# Autodesk Inventor assembly: AGf
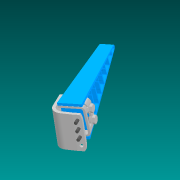
[picture p0: Inventor's stored thumbnail of the model, 180x180]
Saved by Autodesk Inventor 2020.3 (Build 243373000, 373)
## iProperties
Created: 2020-05-25
Part Number: AGf
Document SubType Name: Assembly
Designer: Svend
Author: Svend
## Documents named in this file (4)
- C:\Users\Svend\OneDrive\Documents\GitHub\BeerMinder\3D-model\gripper\AGf.iam
- C:\Users\Svend\OneDrive\Documents\GitHub\BeerMinder\3D-model\servo\AIS2020\3899099 DHAS-MA-B6-80.iam
- C:\Users\Svend\OneDrive\Documents\GitHub\BeerMinder\3D-model\servo\AIS2020\4463570 DHAS-ME-H9-80.iam
- C:\Users\Svend\OneDrive\Documents\GitHub\BeerMinder\3D-model\servo\3998964 DHAS-GF-80-U-BU.ipt
## Components (3 placed, 3 different names)
1. 3899099 DHAS-MA-B6-80:1 [sub-assembly] — Mate:1, Mate:2, Mate:3
2. 4463570 DHAS-ME-H9-80:1 [sub-assembly] — Mate:1, Mate:2, Mate:3, Angle:1, Mate:5, Mate:6, Mate:7
3. 3998964 DHAS-GF-80-U-BU:1 — Angle:1, Mate:5, Mate:6, Mate:7
## Relationships (7: Mate 6, Angle 1)
- Mate:1: 3899099 DHAS-MA-B6-80:1 ↔ 4463570 DHAS-ME-H9-80:1
- Mate:2: 3899099 DHAS-MA-B6-80:1 ↔ 4463570 DHAS-ME-H9-80:1
- Mate:3: 3899099 DHAS-MA-B6-80:1 ↔ 4463570 DHAS-ME-H9-80:1
- Angle:1 (0 deg): 4463570 DHAS-ME-H9-80:1 ↔ 3998964 DHAS-GF-80-U-BU:1
- Mate:5: 4463570 DHAS-ME-H9-80:1 ↔ 3998964 DHAS-GF-80-U-BU:1
- Mate:6: 4463570 DHAS-ME-H9-80:1 ↔ 3998964 DHAS-GF-80-U-BU:1
- Mate:7 (0.2 mm): 4463570 DHAS-ME-H9-80:1 ↔ 3998964 DHAS-GF-80-U-BU:1
